# Autodesk Inventor assembly: T2601_EG
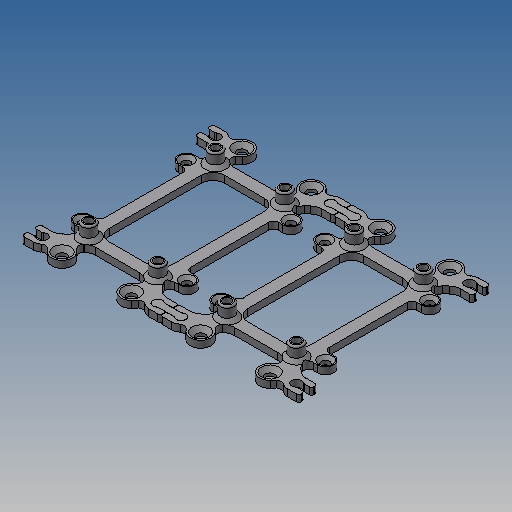
[picture p0: Inventor's stored thumbnail of the model, 512x512]
Saved by Autodesk Inventor 2025.3 (Build 293356000, 356)
## iProperties
Created: 2026-09-18
Part Number: T2601_EG
Project: Nom Projet
Description: Ens. Nom Ensemble
Document SubType Name: Assembly
Designer: jules
Mass: 0.0391901 g
Surface Area: 947.803 cm^2
Volume: 39.1901 cm^3
Density: 0.001 g/cm^3
Author: jules
## Documents named in this file (4)
- C:\Users\jules\OneDrive\PCB_Perso\T2601_APIArduino\T2601_Mecanique\T2601_EG.iam
- C:\Users\jules\OneDrive\PCB_Perso\T2601_APIArduino\T2601_Mecanique\T2601_ExtentionBoard\T2601_ExtentionBoard\T2601_ExtentionBoard.iam
- C:\Users\jules\OneDrive\PCB_Perso\T2601_APIArduino\T2601_Mecanique\T2601_BaseP30.ipt
- C:\Users\jules\OneDrive\PCB_Perso\T2601_APIArduino\T2601_Mecanique\T2601_Conn.ipt
## Components (6 placed, 3 different names)
1. T2601_ExtentionBoard:1 [sub-assembly] — Placage:1, Placage:2, Placage:3
2. T2601_BaseP30:1 — Placage:1, Placage:2, Placage:3, Affleurement:1, Placage:4, Affleurement:2, Angle:1, Placage:7, Affleurement:5
3. T2601_Conn:1 — Placage:6, Placage:7, Affleurement:4
4. T2601_Conn:2 — Placage:4, Placage:5, Affleurement:2, Affleurement:3
5. T2601_BaseP30:2 — Affleurement:1, Placage:5, Affleurement:3, Angle:1, Placage:6, Affleurement:4, Affleurement:5, Placage:8, Placage:9, Placage:10
6. T2601_ExtentionBoard:2 [sub-assembly] — Placage:8, Placage:9, Placage:10
## Relationships (16: Mate 10, Flush 5, Angle 1)
- Placage:1 [Mate]: T2601_ExtentionBoard:1 ↔ T2601_BaseP30:1
- Placage:2 [Mate]: T2601_ExtentionBoard:1 ↔ T2601_BaseP30:1
- Placage:3 [Mate]: T2601_ExtentionBoard:1 ↔ T2601_BaseP30:1
- Affleurement:1 [Flush]: T2601_BaseP30:1 ↔ T2601_BaseP30:2
- Placage:4 [Mate]: T2601_BaseP30:1 ↔ T2601_Conn:2
- Placage:5 [Mate]: T2601_Conn:2 ↔ T2601_BaseP30:2
- Affleurement:2 [Flush]: T2601_BaseP30:1 ↔ T2601_Conn:2
- Affleurement:3 [Flush]: T2601_Conn:2 ↔ T2601_BaseP30:2
- Angle:1 (0 deg): T2601_BaseP30:1 ↔ T2601_BaseP30:2
- Placage:6 [Mate]: T2601_Conn:1 ↔ T2601_BaseP30:2
- Placage:7 [Mate]: T2601_BaseP30:1 ↔ T2601_Conn:1
- Affleurement:4 [Flush]: T2601_Conn:1 ↔ T2601_BaseP30:2
- Affleurement:5 [Flush]: T2601_BaseP30:1 ↔ T2601_BaseP30:2
- Placage:8 [Mate]: T2601_BaseP30:2 ↔ T2601_ExtentionBoard:2
- Placage:9 [Mate]: T2601_BaseP30:2 ↔ T2601_ExtentionBoard:2
- Placage:10 [Mate]: T2601_BaseP30:2 ↔ T2601_ExtentionBoard:2
